# Autodesk Inventor assembly: nsmb_normal
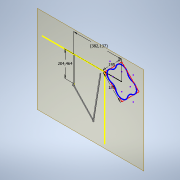
[picture p0: Inventor's stored thumbnail of the model, 180x180]
Saved by Autodesk Inventor 2021 (Build 250183000, 183)
## iProperties
Created: 2021-07-12
Part Number: nsmb_normal
Document SubType Name: Assembly
Designer: Leonardo Fabio Mercado Benítez
Author: Leonardo Fabio Mercado Benítez
## Documents named in this file (5)
- C:\Users\leo7s\Documents\Universidad\02 Servomecanismos\07 Proyecto Final\proyecto_final_Servomecanismos\02 CADs\nsmb_normal.iam
- C:\Users\leo7s\Documents\Universidad\02 Servomecanismos\07 Proyecto Final\proyecto_final_Servomecanismos\02 CADs\trebol_peor_caso_2.ipt
- C:\Users\leo7s\Documents\Universidad\02 Servomecanismos\07 Proyecto Final\proyecto_final_Servomecanismos\02 CADs\base.ipt
- C:\Users\leo7s\Documents\Universidad\02 Servomecanismos\07 Proyecto Final\proyecto_final_Servomecanismos\02 CADs\eslabon_1.ipt
- C:\Users\leo7s\Documents\Universidad\02 Servomecanismos\07 Proyecto Final\proyecto_final_Servomecanismos\02 CADs\eslasbon_2.ipt
## Components (4 placed, 4 different names)
1. trebol_peor_caso_2:1 — Coincidencia:1
2. base:1 — Coincidencia:2, Coincidencia:3, Coincidencia:4
3. eslabon_1:1 — Coincidencia:3, Coincidencia:4, Coincidencia:5, Coincidencia:6
4. eslasbon_2:1 — Coincidencia:5, Coincidencia:6
## Relationships (6: Mate 6)
- Coincidencia:1 [Mate]: trebol_peor_caso_2:1
- Coincidencia:2 [Mate]: base:1
- Coincidencia:3 [Mate]: base:1 ↔ eslabon_1:1
- Coincidencia:4 [Mate]: base:1 ↔ eslabon_1:1
- Coincidencia:5 [Mate]: eslabon_1:1 ↔ eslasbon_2:1
- Coincidencia:6 [Mate]: eslabon_1:1 ↔ eslasbon_2:1
